# Autodesk Inventor assembly: Ensamblaje1
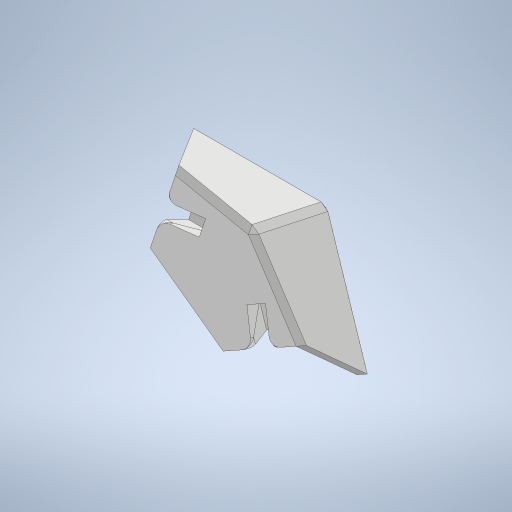
[picture p0: Inventor's stored thumbnail of the model, 512x512]
Saved by Autodesk Inventor 2024 (Build 280153000, 153)
## iProperties
Created: 2025-08-12
Part Number: Ensamblaje1
Document SubType Name: Assembly
Designer: sergi
Author: sergi
## Documents named in this file (4)
- C:\Users\sergi\OneDrive\Escritorio\Ensamblaje1.iam
- C:\Users\sergi\OneDrive\Escritorio\Pieza2.ipt
- C:\Users\sergi\OneDrive\Escritorio\Pieza5.ipt
- C:\Users\sergi\OneDrive\Escritorio\Pieza6.ipt
## Components (9 placed, 3 different names)
1. Pieza2:1 — Coincidencia:4, Coincidencia:5, Coincidencia:6, Nivelación:1, Coincidencia:7
2. Pieza2:2 — Coincidencia:1, Coincidencia:2, Coincidencia:3, Coincidencia:4, Coincidencia:5, Coincidencia:6, Coincidencia:8
3. Pieza2:3 — Coincidencia:1, Coincidencia:2, Coincidencia:3, Coincidencia:10
4. Pieza5:1 — Nivelación:1, Coincidencia:7, Coincidencia:9, Coincidencia:11, Coincidencia:16, Coincidencia:17, Coincidencia:18, Coincidencia:19, Coincidencia:20
5. Pieza5:2 — Coincidencia:8, Coincidencia:9, Coincidencia:12, Coincidencia:13, Coincidencia:15
6. Pieza5:3 — Coincidencia:10, Coincidencia:11, Coincidencia:12, Coincidencia:14
7. Pieza6:1 — Nivelación:2, Nivelación:3
8. Pieza6:2 — Coincidencia:15, Coincidencia:16, Coincidencia:17
9. Pieza6:3 — Coincidencia:18, Coincidencia:19, Coincidencia:20
## Relationships (23: Mate 20, Flush 3)
- Coincidencia:1 [Mate]: Pieza2:2 ↔ Pieza2:3
- Coincidencia:2 [Mate]: Pieza2:2 ↔ Pieza2:3
- Coincidencia:3 [Mate]: Pieza2:2 ↔ Pieza2:3
- Coincidencia:4 [Mate]: Pieza2:1 ↔ Pieza2:2
- Coincidencia:5 [Mate]: Pieza2:1 ↔ Pieza2:2
- Coincidencia:6 [Mate]: Pieza2:1 ↔ Pieza2:2
- Nivelación:1 [Flush]: Pieza2:1 ↔ Pieza5:1
- Coincidencia:7 [Mate]: Pieza2:1 ↔ Pieza5:1
- Coincidencia:8 [Mate]: Pieza2:2 ↔ Pieza5:2
- Coincidencia:9 [Mate]: Pieza5:1 ↔ Pieza5:2
- Coincidencia:10 [Mate]: Pieza2:3 ↔ Pieza5:3
- Coincidencia:11 [Mate]: Pieza5:1 ↔ Pieza5:3
- Coincidencia:12 [Mate]: Pieza5:2 ↔ Pieza5:3
- Coincidencia:13 [Mate]: Pieza5:2
- Coincidencia:14 [Mate]: Pieza5:3
- Nivelación:2 [Flush]: Pieza6:1
- Nivelación:3 [Flush]: Pieza6:1
- Coincidencia:15 [Mate]: Pieza5:2 ↔ Pieza6:2
- Coincidencia:16 [Mate]: Pieza5:1 ↔ Pieza6:2
- Coincidencia:17 [Mate]: Pieza5:1 ↔ Pieza6:2
- Coincidencia:18 [Mate]: Pieza5:1 ↔ Pieza6:3
- Coincidencia:19 [Mate]: Pieza5:1 ↔ Pieza6:3
- Coincidencia:20 [Mate]: Pieza5:1 ↔ Pieza6:3
